# Autodesk Inventor assembly: Splitter with Audio Jacks
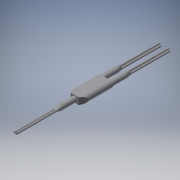
[picture p0: Inventor's stored thumbnail of the model, 180x180]
Saved by Autodesk Inventor 2016 (Build 200138000, 138)
## iProperties
Created: 2015-07-30
Part Number: Splitter with Audio Jacks
Document SubType Name: Assembly
Designer: Nancy
Author: Nancy
## Documents named in this file (3)
- C:\Users\Nancy\Documents\Inventor Files\Splitter with AJ's.iam
- C:\Users\Nancy\Documents\Inventor Files\Male End AJ.ipt
- C:\Users\Nancy\Documents\Inventor Files\Splitter.ipt
## Components (4 placed, 2 different names)
1. Male End AJ:1 — Insert:2
2. Male End AJ:2 — Insert:1, Insert:4
3. Splitter:1 — Insert:1, Insert:2, Insert:3, Insert:4
4. Male End AJ:3 — Insert:3
## Relationships (4: Insert 4)
- Insert:1 (-9.9847 mm): Male End AJ:2 ↔ Splitter:1
- Insert:2 (-15 mm): Male End AJ:1 ↔ Splitter:1
- Insert:3 (-15 mm): Splitter:1 ↔ Male End AJ:3
- Insert:4 (-15 mm): Male End AJ:2 ↔ Splitter:1
